# Autodesk Inventor assembly: Drohne_Mitte
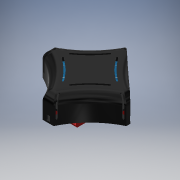
[picture p0: Inventor's stored thumbnail of the model, 180x180]
Saved by Autodesk Inventor 2019 (Build 230136000, 136)
## iProperties
Created: 2018-07-23
Part Number: Drohne_Mitte
Material: Generisch
Document SubType Name: Assembly
Designer: juliu
Author: juliu
## Documents named in this file (7)
- H:\Eule\Bauteile\Mitte\Drohne_Mitte.iam
- H:\Eule\Bauteile\Mitte\grundplatte_oben.ipt
- H:\Eule\Bauteile\Mitte\grundplatte_unten.ipt
- H:\Eule\Bauteile\Mitte\halterung_arm.ipt
- H:\Eule\Bauteile\Mitte\halterung_akku.ipt
- H:\Eule\Bauteile\Mitte\kuppel.ipt
- H:\Eule\Bauteile\Mitte\platine.ipt
## Components (9 placed, 6 different names)
1. grundplatte_unten:1 — Passend:1, Passend:2, Passend:3, Passend:4, Passend:5, Passend:6, Passend:7, Passend:8, Passend:9, Passend:10, Passend:11, Passend:12, Passend:16, Passend:17, Passend:18, Fluchtend:1, Fluchtend:2, Passend:22, Passend:25
2. grundplatte_oben:1 — Passend:13, Passend:14, Passend:15, Passend:19, Passend:20, Passend:21
3. halterung_arm:1 — Passend:4, Passend:7, Passend:8
4. halterung_arm:2 — Passend:3, Passend:5, Passend:6, Passend:13, Passend:14
5. halterung_arm:3 — Passend:2, Passend:11, Passend:12
6. halterung_arm:4 — Passend:1, Passend:9, Passend:10, Passend:15
7. halterung_akku:1 — Passend:16, Passend:17, Passend:18
8. kuppel:1 — Fluchtend:1, Fluchtend:2, Passend:25, Passend:26, Passend:27
9. platine:1 — Passend:19, Passend:20, Passend:21, Passend:23, Passend:24
## Relationships (30: Mate 27, Flush 3)
- Passend:1 [Mate]: grundplatte_unten:1 ↔ halterung_arm:4
- Passend:2 [Mate]: grundplatte_unten:1 ↔ halterung_arm:3
- Passend:3 [Mate]: grundplatte_unten:1 ↔ halterung_arm:2
- Passend:4 [Mate]: grundplatte_unten:1 ↔ halterung_arm:1
- Passend:5 [Mate]: grundplatte_unten:1 ↔ halterung_arm:2
- Passend:6 [Mate]: grundplatte_unten:1 ↔ halterung_arm:2
- Passend:7 [Mate]: grundplatte_unten:1 ↔ halterung_arm:1
- Passend:8 [Mate]: grundplatte_unten:1 ↔ halterung_arm:1
- Passend:9 [Mate]: grundplatte_unten:1 ↔ halterung_arm:4
- Passend:10 [Mate]: grundplatte_unten:1 ↔ halterung_arm:4
- Passend:11 [Mate]: grundplatte_unten:1 ↔ halterung_arm:3
- Passend:12 [Mate]: grundplatte_unten:1 ↔ halterung_arm:3
- Passend:13 [Mate]: grundplatte_oben:1 ↔ halterung_arm:2
- Passend:14 [Mate]: grundplatte_oben:1 ↔ halterung_arm:2
- Passend:15 [Mate]: grundplatte_oben:1 ↔ halterung_arm:4
- Passend:16 [Mate]: grundplatte_unten:1 ↔ halterung_akku:1
- Passend:17 [Mate]: grundplatte_unten:1 ↔ halterung_akku:1
- Passend:18 [Mate]: grundplatte_unten:1 ↔ halterung_akku:1
- Fluchtend:1 [Flush]: grundplatte_unten:1 ↔ kuppel:1
- Fluchtend:2 [Flush]: grundplatte_unten:1 ↔ kuppel:1
- Passend:19 [Mate]: grundplatte_oben:1 ↔ platine:1
- Passend:20 [Mate]: grundplatte_oben:1 ↔ platine:1
- Passend:21 [Mate]: grundplatte_oben:1 ↔ platine:1
- Passend:22 [Mate]: grundplatte_unten:1
- Passend:23 [Mate]: platine:1
- Passend:24 [Mate]: platine:1
- Passend:25 [Mate]: grundplatte_unten:1 ↔ kuppel:1
- Passend:26 [Mate]: kuppel:1
- Passend:27 [Mate]: kuppel:1
- Fluchtend:3 [Flush] (-15 mm)
